# Autodesk Inventor assembly: EsagonoScreeenChiuso
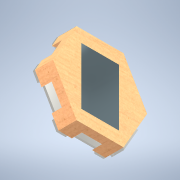
[picture p0: Inventor's stored thumbnail of the model, 180x180]
Saved by Autodesk Inventor 2020 (Build 240168000, 168)
## iProperties
Created: 2020-04-22
Part Number: EsagonoScreeenChiuso
Document SubType Name: Assembly
Designer: Samuele
Author: Samuele
## Documents named in this file (4)
- C:\EsagoniMalsani\ModelliComponenti\EsagonoScreeenChiuso.iam
- C:\EsagoniMalsani\ModelliComponenti\HexagoneBack.ipt
- C:\EsagoniMalsani\ModelliComponenti\Hexagone.ipt
- C:\EsagoniMalsani\ModelliComponenti\TouchLCD.ipt
## Components (3 placed, 3 different names)
1. HexagoneBack:5
2. Hexagone:5 — Flush:9, Mate:8, Mate:9
3. TouchLCD:1 — Flush:9, Mate:8, Mate:9
## Relationships (6: Flush 3, Mate 3)
- [Flush]: HexagoneBack:5 ↔ Hexagone:5
- [Flush]: HexagoneBack:5 ↔ Hexagone:5
- [Mate]: HexagoneBack:5 ↔ Hexagone:5
- Flush:9: Hexagone:5 ↔ TouchLCD:1
- Mate:8: Hexagone:5 ↔ TouchLCD:1
- Mate:9: Hexagone:5 ↔ TouchLCD:1
## Named parameters: d3_d2 = 0 mm, d4_d0 = 0 mm, d5_d1 = 0 mm
